# Autodesk Inventor assembly: End Effector Platform
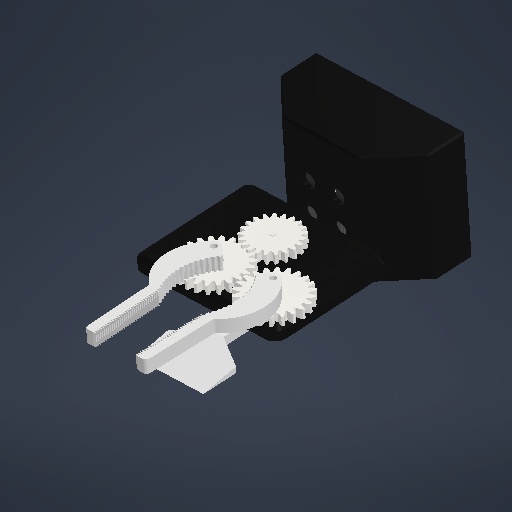
[picture p0: Inventor's stored thumbnail of the model, 512x512]
Saved by Autodesk Inventor 2026.1 (Build 301233000, 233)
## iProperties
Created: 2025-07-17
Part Number: End Effector Platform
Document SubType Name: Assembly
Designer: AdminForWorker
Title: End Effector Platform v38
Author: AdminForWorker
## Documents named in this file (12)
- C:\Users\Sanil\OneDrive\Documents\ENGINEER 1P13\Design Studio\Project 1\teamAssembly 1\End Effector Platform.iam
- C:\Users\Sanil\OneDrive\Documents\ENGINEER 1P13\Design Studio\Project 1\teamAssembly 1\N20 Mini Micro Metall Gear Motor DC 3-6-12V v1 v1.ipt
- C:\Users\Sanil\OneDrive\Documents\ENGINEER 1P13\Design Studio\Project 1\teamAssembly 1\XC-430_idle v3.iam
- C:\Users\Sanil\OneDrive\Documents\ENGINEER 1P13\Design Studio\Project 1\teamAssembly 1\End Effector Platform Base.ipt
- C:\Users\Sanil\OneDrive\Documents\ENGINEER 1P13\Design Studio\Project 1\teamAssembly 1\Quanser QUARC EE Board.ipt
- C:\Users\Sanil\OneDrive\Documents\ENGINEER 1P13\Design Studio\Project 1\teamAssembly 1\End Effector Platform.ipt
- C:\Users\Sanil\OneDrive\Documents\ENGINEER 1P13\Design Studio\Project 1\teamAssembly 1\End Effector Platform Compartment Lid.ipt
- C:\Users\Sanil\OneDrive\Documents\ENGINEER 1P13\Design Studio\Project 1\teamAssembly 1\Gripper Motor Cover.ipt
- C:\Users\Sanil\OneDrive\Documents\ENGINEER 1P13\Design Studio\Project 1\teamAssembly 1\Spur Gear12.ipt
- C:\Users\Sanil\OneDrive\Documents\ENGINEER 1P13\Design Studio\Project 1\teamAssembly 1\Spur Gear14.ipt
- C:\Users\Sanil\OneDrive\Documents\ENGINEER 1P13\Design Studio\Project 1\teamAssembly 1\gripper part.ipt
- C:\Users\Sanil\OneDrive\Documents\ENGINEER 1P13\Design Studio\Project 1\teamAssembly 1\FlatPiece2.ipt
## Components (13 placed, 10 different names)
1. N20 Mini Micro Metall Gear Motor DC 3-6-12V v1 v1:1 — Flush:3, Mate:8, Mate:9, Mate:10, Mate:11, Mate:12, Insert:2
2. XC-430_idle v3:1 [sub-assembly] — Mate:4, Mate:5, Mate:6
3. End Effector Platform Base:1 — Mate:1, Mate:2, Mate:3, Mate:4, Mate:5, Mate:6, Flush:1, Flush:2, Mate:7, Flush:3, Mate:8, Mate:9
4. Quanser QUARC EE Board:1 — Mate:1, Mate:2, Mate:3
5. End Effector Platform:1 — Mate:10, Mate:11, Mate:12, Mate:13, Flush:4, Flush:5, Mate:15, Mate:16, Insert:7, Insert:8
6. End Effector Platform Compartment Lid:1 — Flush:1, Flush:2, Mate:7
7. Gripper Motor Cover:1 — Mate:13, Flush:4, Flush:5
8. Spur Gear1:1 — Insert:2, Rotation:2
9. Spur Gear1:2 — Insert:3, Mate:15, Insert:7, Angle:2, Rotation:1, Insert:9
10. Spur Gear1:3 — Insert:4, Mate:16, Insert:8, Angle:1, Rotation:1, Rotation:2
11. gripper part:1 — Insert:3, Angle:2, Insert:9
12. gripper part:2 — Insert:4, Angle:1
13. FlatPiece2:1
## Relationships (30: Mate 15, Insert 6, Flush 5, Angle 2, RelateRotation 2)
- Mate:1: End Effector Platform Base:1 ↔ Quanser QUARC EE Board:1
- Mate:2: End Effector Platform Base:1 ↔ Quanser QUARC EE Board:1
- Mate:3: End Effector Platform Base:1 ↔ Quanser QUARC EE Board:1
- Mate:4: XC-430_idle v3:1 ↔ End Effector Platform Base:1
- Mate:5: XC-430_idle v3:1 ↔ End Effector Platform Base:1
- Mate:6: XC-430_idle v3:1 ↔ End Effector Platform Base:1
- Flush:1: End Effector Platform Base:1 ↔ End Effector Platform Compartment Lid:1
- Flush:2: End Effector Platform Base:1 ↔ End Effector Platform Compartment Lid:1
- Mate:7: End Effector Platform Base:1 ↔ End Effector Platform Compartment Lid:1
- Flush:3: N20 Mini Micro Metall Gear Motor DC 3-6-12V v1 v1:1 ↔ End Effector Platform Base:1
- Mate:8 (0.2 mm): N20 Mini Micro Metall Gear Motor DC 3-6-12V v1 v1:1 ↔ End Effector Platform Base:1
- Mate:9 (0.2 mm): N20 Mini Micro Metall Gear Motor DC 3-6-12V v1 v1:1 ↔ End Effector Platform Base:1
- Mate:10: N20 Mini Micro Metall Gear Motor DC 3-6-12V v1 v1:1 ↔ End Effector Platform:1
- Mate:11: N20 Mini Micro Metall Gear Motor DC 3-6-12V v1 v1:1 ↔ End Effector Platform:1
- Mate:12: N20 Mini Micro Metall Gear Motor DC 3-6-12V v1 v1:1 ↔ End Effector Platform:1
- Mate:13: End Effector Platform:1 ↔ Gripper Motor Cover:1
- Flush:4: End Effector Platform:1 ↔ Gripper Motor Cover:1
- Flush:5: End Effector Platform:1 ↔ Gripper Motor Cover:1
- Insert:2: N20 Mini Micro Metall Gear Motor DC 3-6-12V v1 v1:1 ↔ Spur Gear1:1
- Insert:3: Spur Gear1:2 ↔ gripper part:1
- Insert:4: Spur Gear1:3 ↔ gripper part:2
- Mate:15: End Effector Platform:1 ↔ Spur Gear1:2
- Mate:16: End Effector Platform:1 ↔ Spur Gear1:3
- Insert:7: End Effector Platform:1 ↔ Spur Gear1:2
- Insert:8: End Effector Platform:1 ↔ Spur Gear1:3
- Angle:1 (90 deg): Spur Gear1:3 ↔ gripper part:2
- Angle:2 (0 deg): Spur Gear1:2 ↔ gripper part:1
- Rotation:1 [RelateRotation] (1 ul): Spur Gear1:2 ↔ Spur Gear1:3
- Rotation:2 [RelateRotation] (1 ul): Spur Gear1:1 ↔ Spur Gear1:3
- Insert:9: Spur Gear1:2 ↔ gripper part:1
